# Autodesk Inventor assembly: Ensamblado general
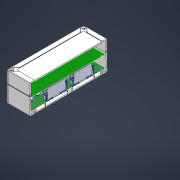
[picture p0: Inventor's stored thumbnail of the model, 180x180]
Saved by Autodesk Inventor 2021 (Build 250183000, 183)
## iProperties
Created: 2022-03-28
Part Number: Ensamblado general
Document SubType Name: Assembly
Designer: Dell
Author: Dell
## Documents named in this file (8)
- C:\Users\Dell\Documents\GitHub\CP_Datalogger\Ensamblado general.iam
- C:\Users\Dell\Documents\GitHub\CP_Datalogger\Enclosure\PowerBoard.iam
- C:\Users\Dell\Documents\GitHub\CP_Datalogger\Enclosure\SpacerWurth970300324.ipt
- C:\Users\Dell\Documents\GitHub\CP_Datalogger\Hardware\LoggerBoard\LoggerBoard.ipt
- C:\Users\Dell\Documents\Inventor\Content Center Files\R2021\en-US\ANSI B18.3.4M(1)\ANSI B18.3.4M - M3 x 0.5 x 3(2).ipt
- C:\Users\Dell\Documents\GitHub\CP_Datalogger\Enclosure\SG22-22B-i.ipt
- C:\Users\Dell\Documents\GitHub\CP_Datalogger\Enclosure\SG-22C-seal-i.ipt
- C:\Users\Dell\Documents\GitHub\CP_Datalogger\Enclosure\SG-22C-i.ipt
## Components (13 placed, 7 different names)
1. PowerBoard:1 [sub-assembly] — Mate:31, Mate:32, Mate:33, Mate:34, Mate:35, Mate:36, Mate:37, Mate:38, Mate:40, Mate:42, Mate:44, Mate:46, Mate:47, Angle:1, Mate:48
2. LoggerBoard:1 — Mate:49, Mate:50, Mate:51
3. SG22-22B-i:1 — Mate:47, Angle:1, Mate:48, Mate:52, Mate:53
4. SG-22C-seal-i:1 — Mate:28, Mate:29, Mate:30
5. SG-22C-i:1 — Mate:28, Mate:29, Mate:30, Mate:52, Mate:53
6. SpacerWurth970300324:1 — Mate:31, Mate:35, Mate:45
7. SpacerWurth970300324:2 — Mate:32, Mate:36, Mate:43, Mate:49
8. SpacerWurth970300324:3 — Mate:33, Mate:37, Mate:39
9. SpacerWurth970300324:4 — Mate:34, Mate:38, Mate:41, Mate:50, Mate:51
10. Broached Hexagon Socket Button Head Cap Screw - Metric M3 x 0.5 x 3:1 — Mate:39, Mate:40
11. Broached Hexagon Socket Button Head Cap Screw - Metric M3 x 0.5 x 3:2 — Mate:41, Mate:42
12. Broached Hexagon Socket Button Head Cap Screw - Metric M3 x 0.5 x 3:3 — Mate:43, Mate:44
13. Broached Hexagon Socket Button Head Cap Screw - Metric M3 x 0.5 x 3:4 — Mate:45, Mate:46
## Relationships (27: Mate 26, Angle 1)
- Mate:28: SG-22C-seal-i:1 ↔ SG-22C-i:1
- Mate:29: SG-22C-seal-i:1 ↔ SG-22C-i:1
- Mate:30: SG-22C-seal-i:1 ↔ SG-22C-i:1
- Mate:31: PowerBoard:1 ↔ SpacerWurth970300324:1
- Mate:32: PowerBoard:1 ↔ SpacerWurth970300324:2
- Mate:33: PowerBoard:1 ↔ SpacerWurth970300324:3
- Mate:34: PowerBoard:1 ↔ SpacerWurth970300324:4
- Mate:35: PowerBoard:1 ↔ SpacerWurth970300324:1
- Mate:36: PowerBoard:1 ↔ SpacerWurth970300324:2
- Mate:37: PowerBoard:1 ↔ SpacerWurth970300324:3
- Mate:38: PowerBoard:1 ↔ SpacerWurth970300324:4
- Mate:39: SpacerWurth970300324:3 ↔ Broached Hexagon Socket Button Head Cap Screw - Metric M3 x 0.5 x 3:1
- Mate:40: PowerBoard:1 ↔ Broached Hexagon Socket Button Head Cap Screw - Metric M3 x 0.5 x 3:1
- Mate:41: SpacerWurth970300324:4 ↔ Broached Hexagon Socket Button Head Cap Screw - Metric M3 x 0.5 x 3:2
- Mate:42: PowerBoard:1 ↔ Broached Hexagon Socket Button Head Cap Screw - Metric M3 x 0.5 x 3:2
- Mate:43: SpacerWurth970300324:2 ↔ Broached Hexagon Socket Button Head Cap Screw - Metric M3 x 0.5 x 3:3
- Mate:44: PowerBoard:1 ↔ Broached Hexagon Socket Button Head Cap Screw - Metric M3 x 0.5 x 3:3
- Mate:45: SpacerWurth970300324:1 ↔ Broached Hexagon Socket Button Head Cap Screw - Metric M3 x 0.5 x 3:4
- Mate:46: PowerBoard:1 ↔ Broached Hexagon Socket Button Head Cap Screw - Metric M3 x 0.5 x 3:4
- Mate:47: PowerBoard:1 ↔ SG22-22B-i:1
- Angle:1 (90 deg): PowerBoard:1 ↔ SG22-22B-i:1
- Mate:48: PowerBoard:1 ↔ SG22-22B-i:1
- Mate:49: LoggerBoard:1 ↔ SpacerWurth970300324:2
- Mate:50: LoggerBoard:1 ↔ SpacerWurth970300324:4
- Mate:51: LoggerBoard:1 ↔ SpacerWurth970300324:4
- Mate:52: SG22-22B-i:1 ↔ SG-22C-i:1
- Mate:53: SG22-22B-i:1 ↔ SG-22C-i:1
